# Autodesk Inventor assembly: Elevatorcarv2
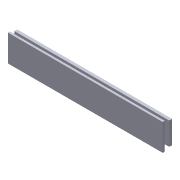
[picture p0: Inventor's stored thumbnail of the model, 180x180]
Saved by Autodesk Inventor 2015 (Build 190159000, 159)
## iProperties
Created: 2015-01-19
Part Number: Elevatorcarv2
Document SubType Name: Assembly
Designer: Tanner
Author: Tanner
## Documents named in this file (4)
- C:\Users\Tanner\Documents\GitHub\FIRST-Team-1719-CAD-Team\2015 Robot CAD\Devices\Elevator and Claw\Elevator Car\Elevator Car.iam
- C:\Users\Tanner\Documents\GitHub\FIRST-Team-1719-CAD-Team\2015 Robot CAD\Devices\Elevator and Claw\Elevator Car\Elevator Car - Bottom.ipt
- C:\Users\Tanner\Documents\GitHub\FIRST-Team-1719-CAD-Team\2015 Robot CAD\Devices\Elevator and Claw\Elevator Car\Elevator Car - BallBearing.ipt
- C:\Users\Tanner\Documents\GitHub\FIRST-Team-1719-CAD-Team\2015 Robot CAD\Devices\Elevator and Claw\Elevator Car\Elevator Car - Top.ipt
## Components (6 placed, 3 different names)
1. Elevator Car - BallBearing:1 — Mate:1, Tangent:2, Tangent:7, Mate:5
2. Elevator Car - BallBearing:2 — Mate:2, Tangent:1, Tangent:6, Tangent:7
3. Elevator Car - BallBearing:3 — Mate:4, Tangent:3, Tangent:8
4. Elevator Car - BallBearing:4 — Mate:3, Tangent:4, Tangent:5, Tangent:8
5. Elevator Car - Bottom:1 — Mate:1, Mate:2, Mate:3, Mate:4, Tangent:1, Tangent:2, Tangent:3, Tangent:4, Tangent:5, Tangent:6, Flush:2, Flush:3
6. Elevator Car - Top:1 — Mate:5, Flush:2, Flush:3
## Relationships (15: Tangent 8, Mate 5, Flush 2)
- Mate:1: Elevator Car - BallBearing:1 ↔ Elevator Car - Bottom:1
- Mate:2: Elevator Car - BallBearing:2 ↔ Elevator Car - Bottom:1
- Mate:3: Elevator Car - BallBearing:4 ↔ Elevator Car - Bottom:1
- Mate:4: Elevator Car - BallBearing:3 ↔ Elevator Car - Bottom:1
- Tangent:1 (6.8326 mm): Elevator Car - BallBearing:2 ↔ Elevator Car - Bottom:1
- Tangent:2 (6.8326 mm): Elevator Car - BallBearing:1 ↔ Elevator Car - Bottom:1
- Tangent:3 (6.8326 mm): Elevator Car - BallBearing:3 ↔ Elevator Car - Bottom:1
- Tangent:4 (6.8326 mm): Elevator Car - BallBearing:4 ↔ Elevator Car - Bottom:1
- Tangent:5 (14.4526 mm): Elevator Car - BallBearing:4 ↔ Elevator Car - Bottom:1
- Tangent:6 (14.4526 mm): Elevator Car - BallBearing:2 ↔ Elevator Car - Bottom:1
- Tangent:7 (16.2052 mm): Elevator Car - BallBearing:1 ↔ Elevator Car - BallBearing:2
- Tangent:8 (16.2052 mm): Elevator Car - BallBearing:3 ↔ Elevator Car - BallBearing:4
- Mate:5: Elevator Car - BallBearing:1 ↔ Elevator Car - Top:1
- Flush:2: Elevator Car - Bottom:1 ↔ Elevator Car - Top:1
- Flush:3 (-3.0353 mm): Elevator Car - Bottom:1 ↔ Elevator Car - Top:1
## Named parameters: noah = 6.8326 mm, tanner = 14.4526 mm, stupid = 16.2052 mm
